# Autodesk Inventor assembly: Ensamblaje
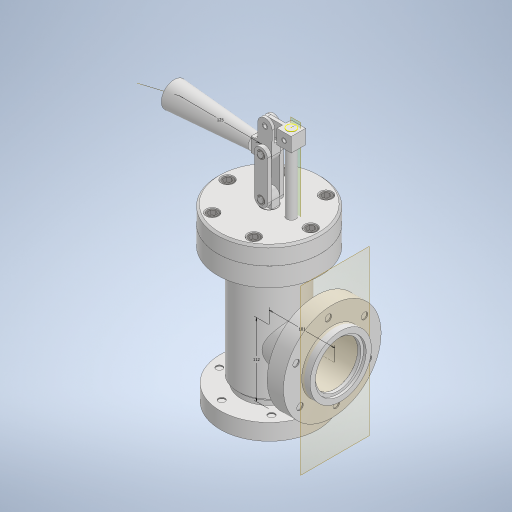
[picture p0: Inventor's stored thumbnail of the model, 512x512]
Saved by Autodesk Inventor 2024.3 (Build 283343000, 343)
## iProperties
Created: 2024-05-16
Part Number: Ensamblaje
Document SubType Name: Assembly
Designer: Cosmic Dinodog
Author: Cosmic Dinodog
## Documents named in this file (21)
- C:\Users\casas\OneDrive\Escritorio\Proyecto DIMAC\Ensamblaje.iam
- C:\Users\casas\OneDrive\Escritorio\Proyecto DIMAC\7_Cuerpo.ipt
- C:\Users\casas\OneDrive\Escritorio\Proyecto DIMAC\6_Piston.ipt
- C:\Users\casas\OneDrive\Escritorio\Proyecto DIMAC\9_AnilloComplementarioA.ipt
- C:\Users\casas\OneDrive\Escritorio\Proyecto DIMAC\20_AnilloPorSoldar2.ipt
- C:\Users\casas\OneDrive\Escritorio\Proyecto DIMAC\3_AnilloPorSoldar.ipt
- C:\Users\casas\OneDrive\Escritorio\Proyecto DIMAC\Resorte.ipt
- C:\Users\casas\OneDrive\Escritorio\Proyecto DIMAC\4_AnilloComplementarioB.ipt
- C:\Users\casas\OneDrive\Escritorio\Proyecto DIMAC\2_VálvulaSuperior.ipt
- C:\Users\casas\OneDrive\Escritorio\Proyecto DIMAC\10_Manija.ipt
- C:\Users\casas\OneDrive\Escritorio\Proyecto DIMAC\19_UnionB.ipt
- C:\Users\casas\OneDrive\Escritorio\Proyecto DIMAC\17_UnionA.ipt
- C:\Users\casas\OneDrive\Escritorio\Proyecto DIMAC\13_Riostra.ipt
- C:\Users\casas\OneDrive\Escritorio\Proyecto DIMAC\12_Pasador.ipt
- C:\Users\casas\OneDrive\Escritorio\Proyecto DIMAC\14_Eje.ipt
- C:\Users\casas\OneDrive\Escritorio\Proyecto DIMAC\16_Soporte.ipt
- C:\Users\casas\OneDrive\Escritorio\Proyecto DIMAC\PasadorResorte.ipt
- C:\Users\casas\OneDrive\Escritorio\Proyecto DIMAC\PasadorExpansion.ipt
- C:\Users\casas\OneDrive\Documentos\Inventor\Content Center Files\R2024\es-ES\ASME B18.27.1 NA1\ASME B18.27.1 NA1 - 3_4.ipt
- C:\Users\casas\OneDrive\Documentos\Inventor\Content Center Files\R2024\es-ES\ASME B18.27.2 NA6\ASME B18.27.2 NA6 - 3_8.ipt
- C:\Users\casas\OneDrive\Documentos\Inventor\Content Center Files\R2024\es-ES\ANSI B18.3.1M(6)\ANSI B18.3.1M - M12x1,75 x 20(1).ipt
## Components (32 placed, 20 different names)
1. 7_Cuerpo:1 — Coincidencia:3, Coincidencia:4, Coincidencia:5, Coincidencia:7, Coincidencia:8, Coincidencia:9, Coincidencia:14
2. 6_Piston:1 — Coincidencia:5, Nivelación:1, Coincidencia:11, Insertar:7
3. 9_AnilloComplementarioA:1 — Coincidencia:1, Coincidencia:2, Coincidencia:3, Coincidencia:4
4. 20_AnilloPorSoldar2:1 — Coincidencia:1, Coincidencia:2
5. 9_AnilloComplementarioA:2 — Coincidencia:7, Coincidencia:10
6. 3_AnilloPorSoldar:1 — Coincidencia:8, Coincidencia:9, Coincidencia:10
7. Resorte:1 — Nivelación:1, Coincidencia:11, Coincidencia:13
8. 20_AnilloPorSoldar2:2 — Coincidencia:12
9. 4_AnilloComplementarioB:1 — Coincidencia:12, Coincidencia:13, Coincidencia:14, Insertar:5, Insertar:6
10. 2_VálvulaSuperior:1 — Insertar:5, Insertar:6, Insertar:8, Insertar:15, Insertar:16, Insertar:17, Insertar:18, Insertar:19, Insertar:20
11. 10_Manija:1 — Insertar:2
12. 19_UnionB:1 — Coincidencia:20, Coincidencia:21, Coincidencia:22, Coincidencia:23, Coincidencia:24, Coincidencia:25, Insertar:2, Insertar:10
13. 17_UnionA:1 — Coincidencia:18, Coincidencia:19, Coincidencia:20, Coincidencia:21, Insertar:9
14. 13_Riostra:1 — Coincidencia:24, Coincidencia:25, Coincidencia:28, Ángulo:1, Insertar:3, Insertar:4, Insertar:13, Insertar:14
15. 13_Riostra:2 — Coincidencia:22, Coincidencia:23, Coincidencia:26, Coincidencia:29, Insertar:11, Insertar:12
16. 12_Pasador:1 — Insertar:4
17. 12_Pasador:2 — Insertar:3
18. 14_Eje:1 — Coincidencia:26, Coincidencia:28, Ángulo:1, Coincidencia:29, Insertar:7, Coincidencia:30, Coincidencia:31
19. 16_Soporte:1 — Coincidencia:18, Coincidencia:19, Insertar:8
20. PasadorResorte:1 — Insertar:9
21. PasadorExpansion:1 — Insertar:10
22. Anillas de retención externas 3/4:1 — Coincidencia:30, Coincidencia:31
23. Anillas de retención externas 3/8:1 — Insertar:11
24. Anillas de retención externas 3/8:2 — Insertar:12
25. Anillas de retención externas 3/8:3 — Insertar:13
26. Anillas de retención externas 3/8:4 — Insertar:14
27. Tornillo forjado de cabeza hueca - Métrico M12x1,75 x 20:1 — Insertar:15
28. Tornillo forjado de cabeza hueca - Métrico M12x1,75 x 20:2 — Insertar:16
29. Tornillo forjado de cabeza hueca - Métrico M12x1,75 x 20:3 — Insertar:17
30. Tornillo forjado de cabeza hueca - Métrico M12x1,75 x 20:4 — Insertar:18
31. Tornillo forjado de cabeza hueca - Métrico M12x1,75 x 20:5 — Insertar:19
32. Tornillo forjado de cabeza hueca - Métrico M12x1,75 x 20:6 — Insertar:20
## Relationships (47: Mate 26, Insert 19, Flush 1, Angle 1)
- Coincidencia:1 [Mate]: 9_AnilloComplementarioA:1 ↔ 20_AnilloPorSoldar2:1
- Coincidencia:2 [Mate]: 9_AnilloComplementarioA:1 ↔ 20_AnilloPorSoldar2:1
- Coincidencia:3 [Mate]: 7_Cuerpo:1 ↔ 9_AnilloComplementarioA:1
- Coincidencia:4 [Mate]: 7_Cuerpo:1 ↔ 9_AnilloComplementarioA:1
- Coincidencia:5 [Mate]: 7_Cuerpo:1 ↔ 6_Piston:1
- Coincidencia:7 [Mate]: 7_Cuerpo:1 ↔ 9_AnilloComplementarioA:2
- Coincidencia:8 [Mate]: 7_Cuerpo:1 ↔ 3_AnilloPorSoldar:1
- Coincidencia:9 [Mate]: 7_Cuerpo:1 ↔ 3_AnilloPorSoldar:1
- Coincidencia:10 [Mate]: 9_AnilloComplementarioA:2 ↔ 3_AnilloPorSoldar:1
- Nivelación:1 [Flush]: 6_Piston:1 ↔ Resorte:1
- Coincidencia:11 [Mate]: 6_Piston:1 ↔ Resorte:1
- Coincidencia:12 [Mate]: 20_AnilloPorSoldar2:2 ↔ 4_AnilloComplementarioB:1
- Coincidencia:13 [Mate]: Resorte:1 ↔ 4_AnilloComplementarioB:1
- Coincidencia:14 [Mate]: 7_Cuerpo:1 ↔ 4_AnilloComplementarioB:1
- Coincidencia:18 [Mate]: 17_UnionA:1 ↔ 16_Soporte:1
- Coincidencia:19 [Mate]: 17_UnionA:1 ↔ 16_Soporte:1
- Coincidencia:20 [Mate]: 19_UnionB:1 ↔ 17_UnionA:1
- Coincidencia:21 [Mate]: 19_UnionB:1 ↔ 17_UnionA:1
- Coincidencia:22 [Mate]: 19_UnionB:1 ↔ 13_Riostra:2
- Coincidencia:23 [Mate]: 19_UnionB:1 ↔ 13_Riostra:2
- Coincidencia:24 [Mate]: 19_UnionB:1 ↔ 13_Riostra:1
- Coincidencia:25 [Mate]: 19_UnionB:1 ↔ 13_Riostra:1
- Coincidencia:26 [Mate]: 13_Riostra:2 ↔ 14_Eje:1
- Coincidencia:28 [Mate]: 13_Riostra:1 ↔ 14_Eje:1
- Ángulo:1 [Angle] (0 deg): 13_Riostra:1 ↔ 14_Eje:1
- Coincidencia:29 [Mate]: 13_Riostra:2 ↔ 14_Eje:1
- Insertar:2: 10_Manija:1 ↔ 19_UnionB:1
- Insertar:3: 13_Riostra:1 ↔ 12_Pasador:2
- Insertar:4: 13_Riostra:1 ↔ 12_Pasador:1
- Insertar:5: 4_AnilloComplementarioB:1 ↔ 2_VálvulaSuperior:1
- Insertar:6: 4_AnilloComplementarioB:1 ↔ 2_VálvulaSuperior:1
- Insertar:7: 6_Piston:1 ↔ 14_Eje:1
- Insertar:8: 2_VálvulaSuperior:1 ↔ 16_Soporte:1
- Insertar:9: 17_UnionA:1 ↔ PasadorResorte:1
- Insertar:10: 19_UnionB:1 ↔ PasadorExpansion:1
- Coincidencia:30 [Mate]: 14_Eje:1 ↔ Anillas de retención externas 3/4:1
- Coincidencia:31 [Mate]: 14_Eje:1 ↔ Anillas de retención externas 3/4:1
- Insertar:11: 13_Riostra:2 ↔ Anillas de retención externas 3/8:1
- Insertar:12: 13_Riostra:2 ↔ Anillas de retención externas 3/8:2
- Insertar:13: 13_Riostra:1 ↔ Anillas de retención externas 3/8:3
- Insertar:14: 13_Riostra:1 ↔ Anillas de retención externas 3/8:4
- Insertar:15: 2_VálvulaSuperior:1 ↔ Tornillo forjado de cabeza hueca - Métrico M12x1,75 x 20:1
- Insertar:16: 2_VálvulaSuperior:1 ↔ Tornillo forjado de cabeza hueca - Métrico M12x1,75 x 20:2
- Insertar:17: 2_VálvulaSuperior:1 ↔ Tornillo forjado de cabeza hueca - Métrico M12x1,75 x 20:3
- Insertar:18: 2_VálvulaSuperior:1 ↔ Tornillo forjado de cabeza hueca - Métrico M12x1,75 x 20:4
- Insertar:19: 2_VálvulaSuperior:1 ↔ Tornillo forjado de cabeza hueca - Métrico M12x1,75 x 20:5
- Insertar:20: 2_VálvulaSuperior:1 ↔ Tornillo forjado de cabeza hueca - Métrico M12x1,75 x 20:6
